# Autodesk Inventor assembly: mainflap
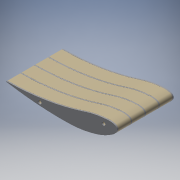
[picture p0: Inventor's stored thumbnail of the model, 180x180]
Saved by Autodesk Inventor 2018 (Build 220112000, 112)
## iProperties
Created: 2018-03-14
Part Number: mainflap
Material: 一般
Document SubType Name: Assembly
Designer: ku_sk
Author: ku_sk
## Documents named in this file (3)
- D:\Users\ku_sk\Documents\Inventor\Aero\KS-15\Rr.wing\parts\mainflap\mainflap.iam
- D:\Users\ku_sk\Documents\Inventor\Aero\KS-15\Rr.wing\parts\mainflap\parts\flap_m.ipt
- D:\Users\ku_sk\Documents\Inventor\Aero\KS-15\Rr.wing\parts\mainflap\parts\uretan_m.ipt
## Components (9 placed, 2 different names)
1. flap_m:1 — メイト:3, メイト:7, メイト:9, メイト:18, メイト:20, メイト:21, メイト:22, メイト:23, メイト:24
2. flap_m:2 — メイト:2, メイト:3, メイト:6, メイト:7, メイト:8, メイト:9, メイト:17
3. flap_m:3 — フラッシュ:1, メイト:1, メイト:2, メイト:4, メイト:6, メイト:8, メイト:10, メイト:11, 角度:1, メイト:15, メイト:16, メイト:19
4. flap_m:4 — メイト:4, メイト:5, メイト:10, メイト:11, メイト:12, メイト:13
5. flap_m:5 — メイト:5, メイト:12, メイト:13, メイト:14
6. uretan_m:1 — メイト:17, メイト:18, メイト:22, メイト:25
7. uretan_m:2 — メイト:16, メイト:20, メイト:23
8. uretan_m:3 — メイト:15, メイト:19, メイト:24
9. uretan_m:4 — メイト:14, メイト:21, メイト:25
## Relationships (27: Mate 25, Flush 1, Angle 1)
- フラッシュ:1 [Flush]: flap_m:3
- メイト:1 [Mate]: flap_m:3
- メイト:2 [Mate] (41.5 mm): flap_m:2 ↔ flap_m:3
- メイト:3 [Mate] (41.5 mm): flap_m:1 ↔ flap_m:2
- メイト:4 [Mate] (41.5 mm): flap_m:3 ↔ flap_m:4
- メイト:5 [Mate] (41.5 mm): flap_m:4 ↔ flap_m:5
- メイト:6 [Mate]: flap_m:2 ↔ flap_m:3
- メイト:7 [Mate]: flap_m:1 ↔ flap_m:2
- メイト:8 [Mate]: flap_m:2 ↔ flap_m:3
- メイト:9 [Mate]: flap_m:1 ↔ flap_m:2
- メイト:10 [Mate]: flap_m:3 ↔ flap_m:4
- メイト:11 [Mate]: flap_m:3 ↔ flap_m:4
- メイト:12 [Mate]: flap_m:4 ↔ flap_m:5
- メイト:13 [Mate]: flap_m:4 ↔ flap_m:5
- 角度:1 [Angle] (0 deg): flap_m:3
- メイト:14 [Mate]: flap_m:5 ↔ uretan_m:4
- メイト:15 [Mate]: flap_m:3 ↔ uretan_m:3
- メイト:16 [Mate]: flap_m:3 ↔ uretan_m:2
- メイト:17 [Mate]: flap_m:2 ↔ uretan_m:1
- メイト:18 [Mate]: flap_m:1 ↔ uretan_m:1
- メイト:19 [Mate]: flap_m:3 ↔ uretan_m:3
- メイト:20 [Mate]: flap_m:1 ↔ uretan_m:2
- メイト:21 [Mate]: flap_m:1 ↔ uretan_m:4
- メイト:22 [Mate]: flap_m:1 ↔ uretan_m:1
- メイト:23 [Mate]: flap_m:1 ↔ uretan_m:2
- メイト:24 [Mate]: flap_m:1 ↔ uretan_m:3
- メイト:25 [Mate]: uretan_m:1 ↔ uretan_m:4
